# Autodesk Inventor assembly: placca
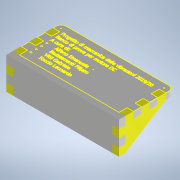
[picture p0: Inventor's stored thumbnail of the model, 180x180]
Saved by Autodesk Inventor 2020.2 (Build 242310000, 310)
## iProperties
Created: 2020-02-13
Part Number: placca
Document SubType Name: Assembly
Designer: socci
Author: socci
## Documents named in this file (4)
- C:\Users\socci\Desktop\placca\placca.iam
- C:\Users\socci\Desktop\placca\base.ipt
- C:\Users\socci\Desktop\placca\sotto.ipt
- C:\Users\socci\Desktop\placca\laterali.ipt
## Components (4 placed, 3 different names)
1. base — Coincidente:1, Allineato:1, Allineato:2, Coincidente:2, Coincidente:5, Allineato:4
2. sotto:1 — Coincidente:1, Allineato:1, Allineato:2, Allineato:3, Coincidente:3, Coincidente:4
3. laterali:1 — Allineato:3, Coincidente:2, Coincidente:3
4. laterali:2 — Coincidente:4, Coincidente:5, Allineato:4
## Relationships (9: Mate 5, Flush 4)
- Coincidente:1 [Mate]: base ↔ sotto:1
- Allineato:1 [Flush]: base ↔ sotto:1
- Allineato:2 [Flush]: base ↔ sotto:1
- Allineato:3 [Flush]: sotto:1 ↔ laterali:1
- Coincidente:2 [Mate]: base ↔ laterali:1
- Coincidente:3 [Mate]: sotto:1 ↔ laterali:1
- Coincidente:4 [Mate]: sotto:1 ↔ laterali:2
- Coincidente:5 [Mate]: base ↔ laterali:2
- Allineato:4 [Flush]: base ↔ laterali:2
